# Autodesk Inventor assembly: boardB
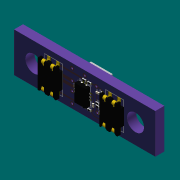
[picture p0: Inventor's stored thumbnail of the model, 180x180]
Saved by Autodesk Inventor 2016 (Build 200138000, 138)
## iProperties
Created: 2016-02-15
Part Number: boardB
Document SubType Name: Assembly
Designer: sawai
Author: sawai
## Documents named in this file (11)
- C:\Users\Sawaiz\OneDrive\projects\mppcSensorInterface\cad\sensorBoardB\boardB.iam
- C:\Users\Sawaiz\OneDrive\projects\mppcSensorInterface\cad\sensorBoardB\pcb.ipt
- C:\Users\Sawaiz\OneDrive\projects\mppcSensorInterface\cad\electronics\788640001\788640001.iam
- C:\Users\Sawaiz\OneDrive\projects\mppcSensorInterface\cad\electronics\udb10LeadQFN3x2.ipt
- C:\Users\Sawaiz\OneDrive\projects\mppcSensorInterface\cad\electronics\chipResistor\chipResistor-0201.ipt
- C:\Users\sawai\OneDrive\projects\mppcSensorInterface\cad\electronics\chipResistor.ipt
- C:\Users\Sawaiz\OneDrive\projects\mppcSensorInterface\cad\electronics\capacitor-0201.ipt
- C:\Users\sawai\OneDrive\projects\mppcSensorInterface\cad\electronics\capacitor.ipt
- C:\Users\Sawaiz\OneDrive\projects\mppcSensorInterface\cad\electronics\L1F2-U.ipt
- C:\Users\Sawaiz\OneDrive\projects\mppcSensorInterface\cad\electronics\chipResistor\chipResistor-0603.ipt
- C:\Users\Sawaiz\OneDrive\projects\mppcSensorInterface\cad\electronics\mppc\MPPC.iam
## Components (20 placed, 8 different names)
1. pcb:1 — Angle:1, Mate:1, Mate:2, Angle:3, Mate:3, Angle:7, Mate:4, Mate:5, Mate:6, Angle:16, Angle:18, Mate:7, Flush:13
2. 788640001:1 [sub-assembly] — Flush:1, Angle:2
3. 788640001:2 [sub-assembly] — Flush:1, Angle:1, Mate:1, Angle:2
4. udb10LeadQFN3x2:1 — Mate:2, Angle:3, Angle:14
5. chipResistor-0201:1 — Flush:2, Angle:4
6. chipResistor-0201:2 — Flush:2, Flush:3, Angle:4, Angle:5, Angle:11
7. chipResistor-0201:3 — Flush:3, Flush:4, Angle:8, Angle:9, Angle:10, Angle:15
8. chipResistor-0201:4 — Flush:4, Flush:5, Angle:9
9. chipResistor-0201:5 — Flush:7, Angle:5, Angle:6
10. chipResistor-0201:6 — Flush:6, Flush:7, Mate:3, Angle:10
11. chipResistor-0201:7 — Flush:5, Flush:6, Angle:6, Angle:7, Angle:8
12. capacitor-0201:1 — Flush:10, Flush:11, Angle:15
13. capacitor-0201:2 — Flush:11, Flush:12, Angle:13
14. capacitor-0201:3 — Flush:12, Angle:13, Angle:14
15. capacitor-0201:4 — Flush:8, Angle:11, Angle:12
16. capacitor-0201:5 — Flush:8, Flush:9, Mate:4, Angle:12
17. capacitor-0201:6 — Flush:9, Flush:10
18. L1F2-U:1 — Mate:5, Angle:17
19. chipResistor-0603:8 — Mate:6, Angle:16, Angle:17
20. MPPC:1 [sub-assembly] — Angle:18, Mate:7, Flush:13
## Relationships (38: Angle 18, Flush 13, Mate 7)
- Flush:1: 788640001:1 ↔ 788640001:2
- Angle:1 (0 deg): pcb:1 ↔ 788640001:2
- Mate:1: pcb:1 ↔ 788640001:2
- Angle:2 (0 deg): 788640001:1 ↔ 788640001:2
- Mate:2: pcb:1 ↔ udb10LeadQFN3x2:1
- Angle:3 (0 deg): pcb:1 ↔ udb10LeadQFN3x2:1
- Flush:2: chipResistor-0201:1 ↔ chipResistor-0201:2
- Flush:3: chipResistor-0201:2 ↔ chipResistor-0201:3
- Flush:4: chipResistor-0201:3 ↔ chipResistor-0201:4
- Flush:5: chipResistor-0201:4 ↔ chipResistor-0201:7
- Flush:6: chipResistor-0201:6 ↔ chipResistor-0201:7
- Flush:7: chipResistor-0201:5 ↔ chipResistor-0201:6
- Mate:3: pcb:1 ↔ chipResistor-0201:6
- Angle:4 (0 deg): chipResistor-0201:1 ↔ chipResistor-0201:2
- Angle:5 (0 deg): chipResistor-0201:2 ↔ chipResistor-0201:5
- Angle:6 (0 deg): chipResistor-0201:5 ↔ chipResistor-0201:7
- Angle:7 (0 deg): pcb:1 ↔ chipResistor-0201:7
- Angle:8 (0 deg): chipResistor-0201:3 ↔ chipResistor-0201:7
- Angle:9 (0 deg): chipResistor-0201:3 ↔ chipResistor-0201:4
- Angle:10 (0 deg): chipResistor-0201:3 ↔ chipResistor-0201:6
- Flush:8: capacitor-0201:4 ↔ capacitor-0201:5
- Flush:9: capacitor-0201:5 ↔ capacitor-0201:6
- Flush:10: capacitor-0201:1 ↔ capacitor-0201:6
- Flush:11: capacitor-0201:1 ↔ capacitor-0201:2
- Flush:12: capacitor-0201:2 ↔ capacitor-0201:3
- Mate:4: pcb:1 ↔ capacitor-0201:5
- Angle:11 (0 deg): chipResistor-0201:2 ↔ capacitor-0201:4
- Angle:12 (0 deg): capacitor-0201:4 ↔ capacitor-0201:5
- Angle:13 (0 deg): capacitor-0201:2 ↔ capacitor-0201:3
- Angle:14 (0 deg): udb10LeadQFN3x2:1 ↔ capacitor-0201:3
- Angle:15 (0 deg): chipResistor-0201:3 ↔ capacitor-0201:1
- Mate:5: pcb:1 ↔ L1F2-U:1
- Mate:6: pcb:1 ↔ chipResistor-0603:8
- Angle:16 (0 deg): pcb:1 ↔ chipResistor-0603:8
- Angle:17 (0 deg): L1F2-U:1 ↔ chipResistor-0603:8
- Angle:18 (0 deg): pcb:1 ↔ MPPC:1
- Mate:7: pcb:1 ↔ MPPC:1
- Flush:13 (10.575 mm): pcb:1 ↔ MPPC:1
